# Autodesk Inventor assembly: Eslabon_motor_L
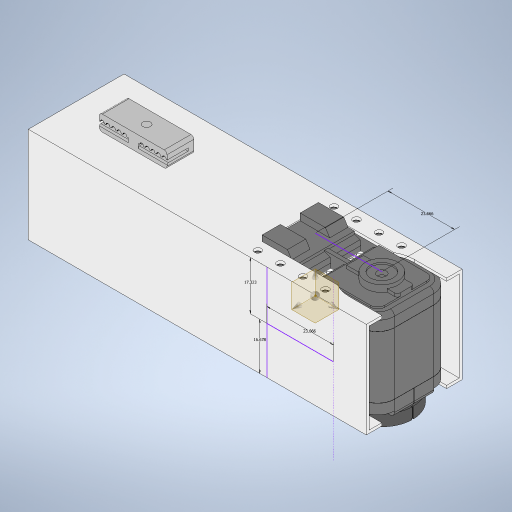
[picture p0: Inventor's stored thumbnail of the model, 512x512]
Saved by Autodesk Inventor 2024 (Build 280153000, 153)
## iProperties
Created: 2023-05-25
Part Number: Eslabon_motor_L
Document SubType Name: Assembly
Designer: epm01
Mass: 61.7407 g
Surface Area: 434.471 cm^2
Volume: 58.246 cm^3
Density: 1.06 g/cm^3
Author: epm01
## Documents named in this file (4)
- D:\Archivos\Inventor\Adaptable\Eslabon_motor_L.iam
- D:\Archivos\Inventor\Adaptable\Eslabon_L.ipt
- D:\Archivos\Inventor\Adaptable\AX-12\AX-12.ipt
- D:\Archivos\Inventor\Banco_pruebas_1\Poleas\coupler\coupler.ipt
## Components (3 placed, 3 different names)
1. Eslabon_L:1 — Coincidencia:1, Coincidencia:2
2. AX-12:1 — Coincidencia:1
3. coupler:1 — Coincidencia:2
## Relationships (2: Mate 2)
- Coincidencia:1 [Mate]: Eslabon_L:1 ↔ AX-12:1
- Coincidencia:2 [Mate]: Eslabon_L:1 ↔ coupler:1
